# Autodesk Inventor assembly: 前脚ギアトレイン5_MIR
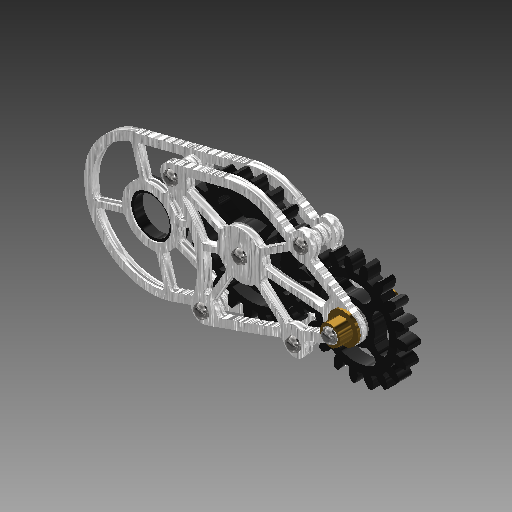
[picture p0: Inventor's stored thumbnail of the model, 512x512]
Saved by Autodesk Inventor 2020 (Build 240168000, 168)
## iProperties
Created: 2019-09-03
Part Number: 前脚ギアトレイン5_MIR
Document SubType Name: Assembly
Designer: 雪村
Mass: 56.2164 g
Surface Area: 264.788 cm^2
Volume: 20.7039 cm^3
Density: 2.71525 g/cm^3
Author: 雪村
## Documents named in this file (11)
- C:\Users\white\Documents\SRDC\SRDC\Inventor_2017\2018年機体\2020年4年機体\前脚ギアトレイン5_MIR.iam
- C:\Users\white\Documents\SRDC\SRDC\Inventor_2017\2018年機体\2020年4年機体\前脚ギアトレイン5.1_MIR.ipt
- C:\Users\white\Documents\SRDC\SRDC\Inventor_2017\2018年機体\2020年4年機体\前脚ギアトレイン5.2_MIR.ipt
- C:\Users\white\Documents\SRDC\SRDC\Inventor_2017\2018年機体\2020年4年機体\歯車m2.z22.ipt
- C:\Users\white\Documents\SRDC\SRDC\Inventor_2017\2018年機体\2020年4年機体\歯車m2.z19.ipt
- C:\Users\white\Documents\SRDC\SRDC\Inventor_2017\2018年機体\パーツ\ベアリングフランジ付き0610.3t.ipt
- C:\Users\white\Documents\SRDC\SRDC\Inventor_2017\2018年機体\パーツ\スペーサーm3,7.ipt
- C:\Users\white\Documents\SRDC\SRDC\Inventor_2017\2018年機体\パーツ\オイレスフランジ付き14162202.5.ipt
- C:\Users\white\Documents\SRDC\SRDC\Inventor_2017\2018年機体\パーツ\オイレスフランジ付き06080512,1t ドライメット.ipt
- C:\Users\white\Documents\SRDC\SRDC\Inventor_2017\2018年機体\パーツ\スペーサーm3,6.ipt
- C:\Users\white\Documents\SRDC\SRDC\Inventor_2017\2018年機体\パーツ\ネジ鍋m3,12.ipt
## Components (26 placed, 10 different names)
1. 前脚ギアトレイン5.1_MIR:1 — 挿入:7, 挿入:8, 挿入:9, 挿入:10, 挿入:11, 挿入:12, 挿入:15, 挿入:16, 挿入:17, 挿入:18, 挿入:19
2. 前脚ギアトレイン5.2_MIR:1 — 挿入:13, 挿入:14, 挿入:20, 挿入:21, 挿入:22, 挿入:23, 挿入:24, 挿入:25, 挿入:26
3. 歯車m2.z22:1
4. 歯車m2.z19:1
5. ベアリングフランジ付き0610.3t:1
6. ベアリングフランジ付き0610.3t:2 — 挿入:10
7. ベアリングフランジ付き0610.3t:3
8. ベアリングフランジ付き0610.3t:4 — 挿入:11
9. スペーサーm3,7:1 — 挿入:18, 挿入:21
10. スペーサーm3,7:2 — 挿入:19, 挿入:20
11. スペーサーm3,7:3 — 挿入:8
12. スペーサーm3,7:4 — 挿入:9
13. スペーサーm3,7:5 — 挿入:17
14. スペーサーm3,7:6 — 挿入:16
15. オイレスフランジ付き14162202.5:1 — 挿入:7
16. オイレスフランジ付き06080512,1t ドライメット:1 — 挿入:15
17. オイレスフランジ付き06080512,1t ドライメット:2 — 挿入:14
18. スペーサーm3,6:1 — 挿入:12
19. スペーサーm3,6:2 — 挿入:13
20. ネジ鍋m3,12:1
21. ネジ鍋m3,12:2
22. ネジ鍋m3,12:5 — 挿入:26
23. ネジ鍋m3,12:6 — 挿入:23
24. ネジ鍋m3,12:7 — 挿入:25
25. ネジ鍋m3,12:8 — 挿入:22
26. ネジ鍋m3,12:9 — 挿入:24
## Relationships (26: Insert 26)
- [Insert]: 歯車m2.z19:1 ↔ ベアリングフランジ付き0610.3t:1
- [Insert]: 歯車m2.z19:1 ↔ ベアリングフランジ付き0610.3t:2
- [Insert]: 歯車m2.z22:1 ↔ ベアリングフランジ付き0610.3t:3
- [Insert]: 歯車m2.z22:1 ↔ ベアリングフランジ付き0610.3t:4
- [Insert]: オイレスフランジ付き06080512,1t ドライメット:1 ↔ ネジ鍋m3,12:1
- [Insert]: スペーサーm3,6:2 ↔ ネジ鍋m3,12:2
- 挿入:7 [Insert]: 前脚ギアトレイン5.1_MIR:1 ↔ オイレスフランジ付き14162202.5:1
- 挿入:8 [Insert]: 前脚ギアトレイン5.1_MIR:1 ↔ スペーサーm3,7:3
- 挿入:9 [Insert]: 前脚ギアトレイン5.1_MIR:1 ↔ スペーサーm3,7:4
- 挿入:10 [Insert]: 前脚ギアトレイン5.1_MIR:1 ↔ ベアリングフランジ付き0610.3t:2
- 挿入:11 [Insert]: 前脚ギアトレイン5.1_MIR:1 ↔ ベアリングフランジ付き0610.3t:4
- 挿入:12 [Insert]: 前脚ギアトレイン5.1_MIR:1 ↔ スペーサーm3,6:1
- 挿入:13 [Insert]: 前脚ギアトレイン5.2_MIR:1 ↔ スペーサーm3,6:2
- 挿入:14 [Insert]: 前脚ギアトレイン5.2_MIR:1 ↔ オイレスフランジ付き06080512,1t ドライメット:2
- 挿入:15 [Insert]: 前脚ギアトレイン5.1_MIR:1 ↔ オイレスフランジ付き06080512,1t ドライメット:1
- 挿入:16 [Insert]: 前脚ギアトレイン5.1_MIR:1 ↔ スペーサーm3,7:6
- 挿入:17 [Insert]: 前脚ギアトレイン5.1_MIR:1 ↔ スペーサーm3,7:5
- 挿入:18 [Insert]: 前脚ギアトレイン5.1_MIR:1 ↔ スペーサーm3,7:1
- 挿入:19 [Insert]: 前脚ギアトレイン5.1_MIR:1 ↔ スペーサーm3,7:2
- 挿入:20 [Insert]: 前脚ギアトレイン5.2_MIR:1 ↔ スペーサーm3,7:2
- 挿入:21 [Insert]: 前脚ギアトレイン5.2_MIR:1 ↔ スペーサーm3,7:1
- 挿入:22 [Insert]: 前脚ギアトレイン5.2_MIR:1 ↔ ネジ鍋m3,12:8
- 挿入:23 [Insert]: 前脚ギアトレイン5.2_MIR:1 ↔ ネジ鍋m3,12:6
- 挿入:24 [Insert]: 前脚ギアトレイン5.2_MIR:1 ↔ ネジ鍋m3,12:9
- 挿入:25 [Insert]: 前脚ギアトレイン5.2_MIR:1 ↔ ネジ鍋m3,12:7
- 挿入:26 [Insert]: 前脚ギアトレイン5.2_MIR:1 ↔ ネジ鍋m3,12:5
